# Autodesk Inventor assembly: Suspensionbogie
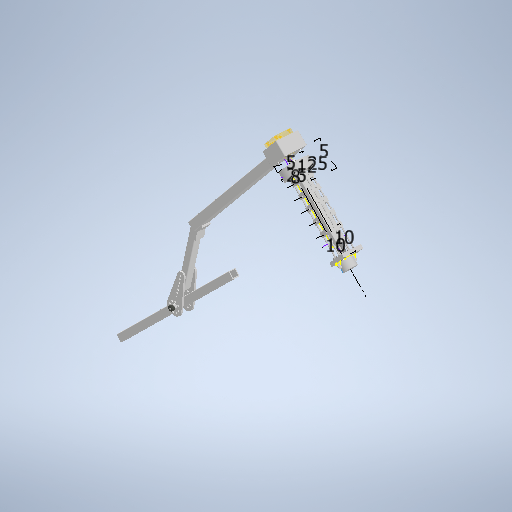
[picture p0: Inventor's stored thumbnail of the model, 512x512]
Saved by Autodesk Inventor 2025.2 (Build 292293000, 293)
## iProperties
Created: 2026-03-19
Part Number: Suspensionbogie
Document SubType Name: Assembly
Designer: hp
Author: hp
## Documents named in this file (32)
- C:\Users\hp\OneDrive\Desktop\Probitymechanicaldocs\Suspensionbogie.iam
- C:\Users\hp\OneDrive\Desktop\Probitymechanicaldocs\Controlarm.ipt
- C:\Users\hp\OneDrive\Desktop\Probitymechanicaldocs\rockershaft.ipt
- C:\Users\hp\OneDrive\Desktop\Probitymechanicaldocs\suspensionarms.ipt
- C:\Users\hp\OneDrive\Desktop\Probitymechanicaldocs\suspensionaxlebearing.ipt
- C:\Users\hp\OneDrive\Desktop\Probitymechanicaldocs\rockerwasher.ipt
- C:\Users\hp\OneDrive\Documents\Inventor\Content Center Files\R2025\en-US\BS EN 24034\ISO 4034 - M6BS EN.ipt
- C:\Users\hp\OneDrive\Documents\Inventor\Content Center Files\R2025\en-US\BS EN 24034\ISO 4034 - M8BS EN.ipt
- C:\Users\hp\OneDrive\Desktop\Probitymechanicaldocs\suspension2chassisarm.ipt
- C:\Users\hp\OneDrive\Desktop\Probitymechanicaldocs\controlarmwasher.ipt
- C:\Users\hp\OneDrive\Documents\Inventor\Content Center Files\R2025\en-US\BS EN ISO 8734\ISO 8734 - 4 x 22BS EN ISO.ipt
- C:\Users\hp\OneDrive\Desktop\Probitymechanicaldocs\150degreebracket.ipt
- C:\Users\hp\OneDrive\Desktop\Probitymechanicaldocs\rockerpivotarm.ipt
- C:\Users\hp\OneDrive\Desktop\Probitymechanicaldocs\turnmotorcasing.ipt
- C:\Users\hp\OneDrive\Desktop\Probitymechanicaldocs\turnmotor.ipt
- C:\Users\hp\OneDrive\Documents\Inventor\Content Center Files\R2025\en-US\ISO 1580\ISO 1580 - M2.5 x 3_.ipt
- C:\Users\hp\OneDrive\Desktop\Probitymechanicaldocs\hexcoupling.ipt
- C:\Users\hp\OneDrive\Documents\Inventor\Content Center Files\R2025\en-US\ISO 1580\ISO 1580 - M1.6 x 2_.ipt
- C:\Users\hp\OneDrive\Desktop\Probitymechanicaldocs\couplingload.ipt
- C:\Users\hp\OneDrive\Desktop\Probitymechanicaldocs\turningthrustbearing.ipt
- C:\Users\hp\OneDrive\Desktop\Probitymechanicaldocs\verticalaxle.ipt
- C:\Users\hp\OneDrive\Desktop\Probitymechanicaldocs\leadscrew.ipt
- C:\Users\hp\OneDrive\Desktop\Probitymechanicaldocs\RISE&Fallmotor.ipt
- C:\Users\hp\OneDrive\Desktop\Probitymechanicaldocs\leadscrewaxle.ipt
- C:\Users\hp\OneDrive\Desktop\Probitymechanicaldocs\sleeve.ipt
- C:\Users\hp\OneDrive\Desktop\Probitymechanicaldocs\placeholderjoint.ipt
- C:\Users\hp\OneDrive\Desktop\Probitymechanicaldocs\impromptugraphitering.ipt
- C:\Users\hp\OneDrive\Desktop\Probitymechanicaldocs\Placeholderjointouterring.ipt
- C:\Users\hp\OneDrive\Desktop\Probitymechanicaldocs\spokes.ipt
- C:\Users\hp\OneDrive\Desktop\Probitymechanicaldocs\liftmotorfloor.ipt
- C:\Users\hp\OneDrive\Documents\Inventor\Content Center Files\R2025\en-US\ISO 4032(2)\ISO 4032 - M4 - ISO.ipt
- C:\Users\hp\OneDrive\Desktop\Probitymechanicaldocs\liftmotorbasenut.ipt
## Components (72 placed, 31 different names)
1. Controlarm:1 — Rotational:6, Rotational:8, Rotational:12, Rotational:13, Rotational:14, Rotational:18
2. rockershaft:1 — Mate:1, Cylindrical:1
3. suspensionarms:1 — Rotational:1, Rotational:2
4. suspensionaxlebearing:1 — Rotational:1, Rotational:3, Cylindrical:1
5. Controlarm:2 — Rotational:5, Rotational:7, Rotational:11, Rotational:15, Rotational:16, Rotational:17
6. suspensionaxlebearing:2 — Rotational:2, Rotational:4
7. rockerwasher:1 — Rotational:4, Rotational:6
8. rockerwasher:2 — Rotational:3, Rotational:5
9. suspensionaxlebearing:3 — Rotational:7, Rotational:9
10. suspensionaxlebearing:4 — Rotational:8, Rotational:10
11. rockerwasher:3 — Rotational:9, Insert:1
12. rockerwasher:4 — Rotational:10, Mate:2
13. BS EN 24034 - Metric M6:1 — Insert:1, Insert:7, Mate:5
14. BS EN 24034 - Metric M8:1 — Mate:1, Mate:2
15. suspension2chassisarm:1 — Rotational:19, Rotational:20, Slider:2
16. controlarmwasher:1 — Rotational:12, Cylindrical:5
17. controlarmwasher:2 — Rotational:11, Rotational:19
18. controlarmwasher:3 — Rotational:18, Rotational:20, Cylindrical:4
19. controlarmwasher:4 — Rotational:15
20. controlarmwasher:5 — Rotational:17
21. controlarmwasher:6 — Rotational:16
22. controlarmwasher:7 — Rotational:13, Cylindrical:2
23. controlarmwasher:8 — Rotational:14, Cylindrical:3
24. BS EN ISO 8734 4 x 22:1 — Insert:2, Cylindrical:2
25. BS EN ISO 8734 4 x 22:2 — Cylindrical:3
26. BS EN ISO 8734 4 x 22:3 — Cylindrical:4
27. BS EN ISO 8734 4 x 22:4 — Cylindrical:5
28. BS EN ISO 8734 4 x 22:5 — Insert:2
29. 150degreebracket:1 — Slider:1, Mate:3, Slider:2
30. rockerpivotarm:1 — Slider:1, Mate:3, Slider:3
31. turnmotorcasing:1 — Slider:3, Rigid:1, Insert:3, Insert:4, Insert:5, Insert:6, Rotational:22
32. turnmotor:1 — Rigid:1, Rotational:21, Angle:1
33. ISO 1580 M2.5 x 3:1 — Insert:3
34. ISO 1580 M2.5 x 3:2 — Insert:4
35. ISO 1580 M2.5 x 3:3 — Insert:5
36. ISO 1580 M2.5 x 3:4 — Insert:6
37. hexcoupling:1 — Rotational:21, Angle:1, Mate:4, Rigid:2
38. ISO 1580 M2.5 x 3:5 — Mate:4
39. ISO 1580 M1.6 x 2:1 — Insert:7, Mate:5
40. couplingload:1 — Rigid:2, Rotational:23
41. turningthrustbearing:1 — Rotational:22
42. verticalaxle:1 — Rotational:23, Mate:6, Mate:7, Rotational:24, Mate:9, Rotational:25, Rotational:26, Rotational:27, Rotational:28, Rotational:29, Rotational:30, Rotational:31, Rotational:32, Rotational:33, Rotational:34, Rotational:35
43. leadscrew:1 — Cylindrical:7, Rotational:24, Mate:9
44. RISE&Fallmotor:1 — Cylindrical:6, Mate:8, Rotational:40, Rotational:41, Rotational:50, Rotational:51
45. leadscrewaxle:1 — Cylindrical:6, Mate:8, Cylindrical:7
46. sleeve:1 — Rotational:25, Rotational:26
47. sleeve:2 — Rotational:27
48. sleeve:3 — Rotational:28, Rotational:29
49. sleeve:4 — Rotational:30, Rotational:31
50. sleeve:5 — Rotational:32, Rotational:33
51. sleeve:6 — Rotational:34, Rotational:35, Rotational:36, Rotational:37, Insert:8
52. placeholderjoint:1 — Rotational:36, Rotational:37, Cylindrical:8
53. impromptugraphitering:1 — Cylindrical:8, Rotational:38, Rotational:39
54. Placeholderjointouterring:1 — Rotational:38
55. Placeholderjointouterring:2 — Rotational:39
56. spokes:1 — Rotational:44
57. spokes:2 — Rotational:45
58. spokes:3 — Rotational:48
59. spokes:4 — Rotational:49
60. spokes:8 — Rotational:46
61. spokes:9 — Rotational:43, Insert:8
62. spokes:11 — Rotational:47
63. spokes:12 — Rotational:42
64. liftmotorfloor:1 — Rotational:40, Rotational:41, Rotational:42, Rotational:43, Rotational:44, Rotational:45, Rotational:46, Rotational:47, Rotational:48, Rotational:49, Mate:10, Mate:11, Mate:12, Mate:13
65. ISO 4032 M4:1 — Mate:10, Mate:11
66. ISO 4032 M4:2 — Mate:12, Mate:13
67. liftmotorbasenut:1 — Rotational:50
68. liftmotorbasenut:2 — Rotational:51
69. ISO 1580 M2.5 x 3:6 — Mate:6, Mate:7
70. ISO 1580 M2.5 x 3:7
71. ISO 1580 M2.5 x 3:8
72. ISO 1580 M2.5 x 3:9
## Component patterns: (4 elements, first: ISO 1580 M2.5 x 3:6)
## Relationships (86: RevoluteJoint 51, Mate 13, Insert 8, CylindricalJoint 8, TranslationJoint 3, WeldJoint 2, Angle 1)
- Rotational:1 [RevoluteJoint]: suspensionarms:1 ↔ suspensionaxlebearing:1
- Rotational:2 [RevoluteJoint]: suspensionarms:1 ↔ suspensionaxlebearing:2
- Rotational:3 [RevoluteJoint]: suspensionaxlebearing:1 ↔ rockerwasher:2
- Rotational:4 [RevoluteJoint]: suspensionaxlebearing:2 ↔ rockerwasher:1
- Rotational:5 [RevoluteJoint]: Controlarm:2 ↔ rockerwasher:2
- Rotational:6 [RevoluteJoint]: Controlarm:1 ↔ rockerwasher:1
- Rotational:7 [RevoluteJoint]: Controlarm:2 ↔ suspensionaxlebearing:3
- Rotational:8 [RevoluteJoint]: Controlarm:1 ↔ suspensionaxlebearing:4
- Rotational:9 [RevoluteJoint]: suspensionaxlebearing:3 ↔ rockerwasher:3
- Rotational:10 [RevoluteJoint]: suspensionaxlebearing:4 ↔ rockerwasher:4
- Insert:1: rockerwasher:3 ↔ BS EN 24034 - Metric M6:1
- Mate:1: rockershaft:1 ↔ BS EN 24034 - Metric M8:1
- Mate:2: rockerwasher:4 ↔ BS EN 24034 - Metric M8:1
- Cylindrical:1: rockershaft:1 ↔ suspensionaxlebearing:1
- Rotational:11 [RevoluteJoint]: Controlarm:2 ↔ controlarmwasher:2
- Rotational:12 [RevoluteJoint]: Controlarm:1 ↔ controlarmwasher:1
- Rotational:13 [RevoluteJoint]: Controlarm:1 ↔ controlarmwasher:7
- Rotational:14 [RevoluteJoint]: Controlarm:1 ↔ controlarmwasher:8
- Rotational:15 [RevoluteJoint]: Controlarm:2 ↔ controlarmwasher:4
- Rotational:16 [RevoluteJoint]: Controlarm:2 ↔ controlarmwasher:6
- Rotational:17 [RevoluteJoint]: Controlarm:2 ↔ controlarmwasher:5
- Rotational:18 [RevoluteJoint]: Controlarm:1 ↔ controlarmwasher:3
- Rotational:19 [RevoluteJoint]: suspension2chassisarm:1 ↔ controlarmwasher:2
- Rotational:20 [RevoluteJoint]: suspension2chassisarm:1 ↔ controlarmwasher:3
- Insert:2: BS EN ISO 8734 4 x 22:1 ↔ BS EN ISO 8734 4 x 22:5
- Cylindrical:2: controlarmwasher:7 ↔ BS EN ISO 8734 4 x 22:1
- Cylindrical:3: controlarmwasher:8 ↔ BS EN ISO 8734 4 x 22:2
- Cylindrical:4: controlarmwasher:3 ↔ BS EN ISO 8734 4 x 22:3
- Cylindrical:5: controlarmwasher:1 ↔ BS EN ISO 8734 4 x 22:4
- Slider:1 [TranslationJoint]: 150degreebracket:1 ↔ rockerpivotarm:1
- Mate:3 (28 mm): 150degreebracket:1 ↔ rockerpivotarm:1
- Slider:2 [TranslationJoint]: suspension2chassisarm:1 ↔ 150degreebracket:1
- Slider:3 [TranslationJoint]: rockerpivotarm:1 ↔ turnmotorcasing:1
- Rigid:1 [WeldJoint]: turnmotorcasing:1 ↔ turnmotor:1
- Insert:3: turnmotorcasing:1 ↔ ISO 1580 M2.5 x 3:1
- Insert:4: turnmotorcasing:1 ↔ ISO 1580 M2.5 x 3:2
- Insert:5: turnmotorcasing:1 ↔ ISO 1580 M2.5 x 3:3
- Insert:6: turnmotorcasing:1 ↔ ISO 1580 M2.5 x 3:4
- Rotational:21 [RevoluteJoint]: turnmotor:1 ↔ hexcoupling:1
- Angle:1 (0 deg): turnmotor:1 ↔ hexcoupling:1
- Mate:4: hexcoupling:1 ↔ ISO 1580 M2.5 x 3:5
- Insert:7: BS EN 24034 - Metric M6:1 ↔ ISO 1580 M1.6 x 2:1
- Mate:5: BS EN 24034 - Metric M6:1 ↔ ISO 1580 M1.6 x 2:1
- Rigid:2 [WeldJoint]: hexcoupling:1 ↔ couplingload:1
- Rotational:22 [RevoluteJoint]: turnmotorcasing:1 ↔ turningthrustbearing:1
- Rotational:23 [RevoluteJoint]: couplingload:1 ↔ verticalaxle:1
- Mate:6: verticalaxle:1 ↔ ISO 1580 M2.5 x 3:6
- Mate:7: verticalaxle:1 ↔ ISO 1580 M2.5 x 3:6
- Cylindrical:6: RISE&Fallmotor:1 ↔ leadscrewaxle:1
- Mate:8: RISE&Fallmotor:1 ↔ leadscrewaxle:1
- Cylindrical:7: leadscrew:1 ↔ leadscrewaxle:1
- Rotational:24 [RevoluteJoint]: verticalaxle:1 ↔ leadscrew:1
- Mate:9: verticalaxle:1 ↔ leadscrew:1
- Rotational:25 [RevoluteJoint]: verticalaxle:1 ↔ sleeve:1
- Rotational:26 [RevoluteJoint]: verticalaxle:1 ↔ sleeve:1
- Rotational:27 [RevoluteJoint]: verticalaxle:1 ↔ sleeve:2
- Rotational:28 [RevoluteJoint]: verticalaxle:1 ↔ sleeve:3
- Rotational:29 [RevoluteJoint]: verticalaxle:1 ↔ sleeve:3
- Rotational:30 [RevoluteJoint]: verticalaxle:1 ↔ sleeve:4
- Rotational:31 [RevoluteJoint]: verticalaxle:1 ↔ sleeve:4
- Rotational:32 [RevoluteJoint]: verticalaxle:1 ↔ sleeve:5
- Rotational:33 [RevoluteJoint]: verticalaxle:1 ↔ sleeve:5
- Rotational:34 [RevoluteJoint]: verticalaxle:1 ↔ sleeve:6
- Rotational:35 [RevoluteJoint]: verticalaxle:1 ↔ sleeve:6
- Rotational:36 [RevoluteJoint]: sleeve:6 ↔ placeholderjoint:1
- Rotational:37 [RevoluteJoint]: sleeve:6 ↔ placeholderjoint:1
- Cylindrical:8: placeholderjoint:1 ↔ impromptugraphitering:1
- Rotational:38 [RevoluteJoint]: impromptugraphitering:1 ↔ Placeholderjointouterring:1
- Rotational:39 [RevoluteJoint]: impromptugraphitering:1 ↔ Placeholderjointouterring:2
- Rotational:40 [RevoluteJoint]: RISE&Fallmotor:1 ↔ liftmotorfloor:1
- Rotational:41 [RevoluteJoint]: RISE&Fallmotor:1 ↔ liftmotorfloor:1
- Rotational:42 [RevoluteJoint]: spokes:12 ↔ liftmotorfloor:1
- Rotational:43 [RevoluteJoint]: spokes:9 ↔ liftmotorfloor:1
- Rotational:44 [RevoluteJoint]: spokes:1 ↔ liftmotorfloor:1
- Rotational:45 [RevoluteJoint]: spokes:2 ↔ liftmotorfloor:1
- Rotational:46 [RevoluteJoint]: spokes:8 ↔ liftmotorfloor:1
- Rotational:47 [RevoluteJoint]: spokes:11 ↔ liftmotorfloor:1
- Rotational:48 [RevoluteJoint]: spokes:3 ↔ liftmotorfloor:1
- Rotational:49 [RevoluteJoint]: spokes:4 ↔ liftmotorfloor:1
- Insert:8: sleeve:6 ↔ spokes:9
- Mate:10: liftmotorfloor:1 ↔ ISO 4032 M4:1
- Mate:11: liftmotorfloor:1 ↔ ISO 4032 M4:1
- Mate:12: liftmotorfloor:1 ↔ ISO 4032 M4:2
- Mate:13: liftmotorfloor:1 ↔ ISO 4032 M4:2
- Rotational:50 [RevoluteJoint]: RISE&Fallmotor:1 ↔ liftmotorbasenut:1
- Rotational:51 [RevoluteJoint]: RISE&Fallmotor:1 ↔ liftmotorbasenut:2
